# Autodesk Inventor assembly: Motor and Bracket for Rack and Pinion
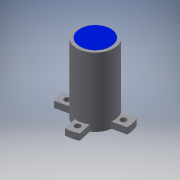
[picture p0: Inventor's stored thumbnail of the model, 180x180]
Saved by Autodesk Inventor 2016 (Build 200138000, 138)
## iProperties
Created: 2016-04-18
Part Number: Motor and Bracket for Rack and Pinion
Document SubType Name: Assembly
Designer: Andrea
Author: Andrea
## Documents named in this file (3)
- C:\Users\Andrea\Documents\Dropbox\Capstone CAD\Motor + Attachment\Motor and Bracket for Rack and Pinion.iam
- C:\Users\Andrea\Documents\Dropbox\Capstone CAD\Motor Mount Rack and Pinion.ipt
- C:\Users\Andrea\Documents\Dropbox\Capstone CAD\Motor + Attachment\Motor + Shaft.iam
## Components (2 placed, 2 different names)
1. Motor Mount Rack and Pinion:1 — Mate:1, Mate:2
2. Motor + Shaft:1 [sub-assembly] — Mate:1, Mate:2
## Relationships (2: Mate 2)
- Mate:1: Motor Mount Rack and Pinion:1 ↔ Motor + Shaft:1
- Mate:2: Motor Mount Rack and Pinion:1 ↔ Motor + Shaft:1
